# Autodesk Inventor assembly: Robot Ensamblado
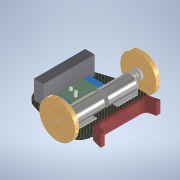
[picture p0: Inventor's stored thumbnail of the model, 180x180]
Saved by Autodesk Inventor 2022.2 (Build 262287010, 287A)
## iProperties
Created: 2022-03-28
Part Number: Robot Ensamblado
Document SubType Name: Assembly
Designer: Santiago Larraín
Author: Santiago Larraín
## Documents named in this file (11)
- C:\Users\Santiago Larraín\Documents\Archivos  PUC\5to Semestre 2022\Fundamentos de la Robótica\Tarea 1\Nuevos Diseños\Robot Ensamblado.iam
- C:\Users\Santiago Larraín\Documents\Archivos  PUC\5to Semestre 2022\Fundamentos de la Robótica\Tarea 1\Nuevos Diseños\Base del Robot.ipt
- C:\Users\Santiago Larraín\Documents\Archivos  PUC\5to Semestre 2022\Fundamentos de la Robótica\Tarea 1\Piezas 3D Robot - Simplificado\LBracket.ipt
- C:\Users\Santiago Larraín\Documents\Archivos  PUC\5to Semestre 2022\Fundamentos de la Robótica\Tarea 1\Piezas 3D Robot - Simplificado\Gearmotor.ipt
- C:\Users\Santiago Larraín\Documents\Archivos  PUC\5to Semestre 2022\Fundamentos de la Robótica\Tarea 1\Piezas 3D Robot - Simplificado\MountingHub.ipt
- C:\Users\Santiago Larraín\Documents\Archivos  PUC\5to Semestre 2022\Fundamentos de la Robótica\Tarea 1\Piezas 3D Robot - Simplificado\Wheel.ipt
- C:\Users\Santiago Larraín\Documents\Archivos  PUC\5to Semestre 2022\Fundamentos de la Robótica\Tarea 1\Piezas 3D Robot - Simplificado\ArduinoMega.ipt
- C:\Users\Santiago Larraín\Documents\Archivos  PUC\5to Semestre 2022\Fundamentos de la Robótica\Tarea 1\Piezas 3D Robot - Simplificado\MotorDriverShield.ipt
- C:\Users\Santiago Larraín\Documents\Archivos  PUC\5to Semestre 2022\Fundamentos de la Robótica\Tarea 1\Piezas 3D Robot - Simplificado\Bateria.ipt
- C:\Users\Santiago Larraín\Documents\Archivos  PUC\5to Semestre 2022\Fundamentos de la Robótica\Tarea 1\Piezas 3D Robot - Simplificado\BackWheel.ipt
- C:\Users\Santiago Larraín\Documents\Archivos  PUC\5to Semestre 2022\Fundamentos de la Robótica\Tarea 1\Nuevos Diseños\Pala del Robot.ipt
## Components (14 placed, 10 different names)
1. Base del Robot:1 — Mate:1, Mate:2, Mate:3, Mate:5, Tangent:1, Mate:6
2. LBracket:1 — Insert:1, Mate:2
3. Gearmotor:2 — Insert:1, Insert:2, Insert:7
4. MountingHub:1 — Insert:2, Insert:3
5. Wheel:1 — Insert:3
6. LBracket:2 — Mate:1
7. Gearmotor:3 — Insert:7
8. MountingHub:2
9. Wheel:2
10. ArduinoMega:1 — Mate:3, Mate:4
11. MotorDriverShield:1 — Mate:4
12. Bateria:1 — Mate:5
13. BackWheel:1 — Tangent:1
14. Pala del Robot:1 — Mate:6
## Relationships (14: Insert 7, Mate 6, Tangent 1)
- Insert:1: LBracket:1 ↔ Gearmotor:2
- Insert:2: Gearmotor:2 ↔ MountingHub:1
- Insert:3: MountingHub:1 ↔ Wheel:1
- [Insert]: LBracket:2 ↔ Gearmotor:3
- [Insert]: Gearmotor:3 ↔ MountingHub:2
- [Insert]: MountingHub:2 ↔ Wheel:2
- Mate:1: Base del Robot:1 ↔ LBracket:2
- Mate:2: Base del Robot:1 ↔ LBracket:1
- Insert:7 (10 mm): Gearmotor:2 ↔ Gearmotor:3
- Mate:3: Base del Robot:1 ↔ ArduinoMega:1
- Mate:4: ArduinoMega:1 ↔ MotorDriverShield:1
- Mate:5: Base del Robot:1 ↔ Bateria:1
- Tangent:1: Base del Robot:1 ↔ BackWheel:1
- Mate:6: Base del Robot:1 ↔ Pala del Robot:1
## Named parameters: d4_d1 = 0 mm, d5_d2 = 0 mm, d6_d3 = 0 mm
